# Autodesk Inventor assembly: 13_centerlegg_assembly
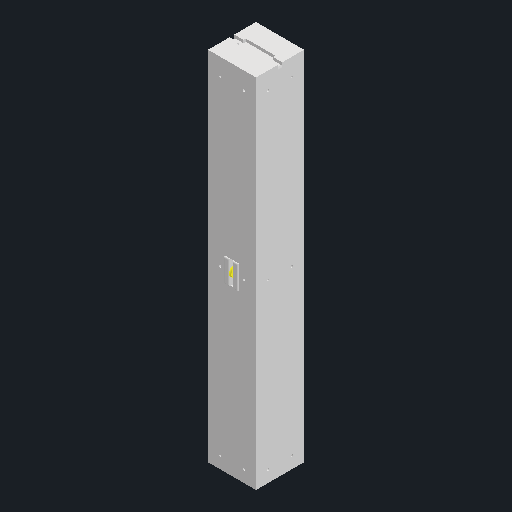
[picture p0: Inventor's stored thumbnail of the model, 512x512]
Saved by Autodesk Inventor 2024 (Build 280153000, 153)
## iProperties
Created: 2023-05-24
Part Number: 13_centerlegg_assembly
Document SubType Name: Assembly
Designer: aasmu
Author: aasmu
## Documents named in this file (6)
- C:\Users\aasmu\Documents\standing_desk\13_centerlegg_assembly.iam
- C:\Users\aasmu\Documents\standing_desk\07_centerlegg_short_side.ipt
- C:\Users\aasmu\Documents\standing_desk\centerlegg_long_side.ipt
- C:\Users\aasmu\Documents\standing_desk\inner_glide_carriage\10_inner_glide_carriage_assembly.iam
- C:\Users\aasmu\Documents\standing_desk\inner_glide_carriage\11_inner_glide_carriage_roller_assembly.iam
- C:\Users\aasmu\Documents\standing_desk\09_centerlegg_topplate.ipt
## Components (8 placed, 5 different names)
1. 07_centerlegg_short_side:1 — Rigid:2
2. 07_centerlegg_short_side:2 — Rigid:1, Rigid:5
3. centerlegg_long_side:1 — Rigid:6
4. centerlegg_long_side:2 — Rigid:3, Rigid:4, Rigid:7
5. 10_inner_glide_carriage_assembly:1 [sub-assembly] — Rigid:4, Rigid:6
6. 10_inner_glide_carriage_assembly:2 [sub-assembly] — Rigid:1, Rigid:2, Rigid:3
7. 11_inner_glide_carriage_roller_assembly:1 [sub-assembly] — Rigid:5
8. 09_centerlegg_topplate:1 — Rigid:7
## Relationships (7: WeldJoint 7)
- Rigid:1 [WeldJoint]: 07_centerlegg_short_side:2 ↔ 10_inner_glide_carriage_assembly:2
- Rigid:2 [WeldJoint]: 07_centerlegg_short_side:1 ↔ 10_inner_glide_carriage_assembly:2
- Rigid:3 [WeldJoint]: centerlegg_long_side:2 ↔ 10_inner_glide_carriage_assembly:2
- Rigid:4 [WeldJoint]: centerlegg_long_side:2 ↔ 10_inner_glide_carriage_assembly:1
- Rigid:5 [WeldJoint]: 07_centerlegg_short_side:2 ↔ 11_inner_glide_carriage_roller_assembly:1
- Rigid:6 [WeldJoint]: centerlegg_long_side:1 ↔ 10_inner_glide_carriage_assembly:1
- Rigid:7 [WeldJoint]: centerlegg_long_side:2 ↔ 09_centerlegg_topplate:1
